# Autodesk Inventor assembly: 100-CHASSIS-ASM-01
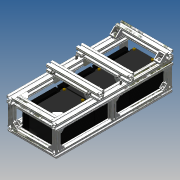
[picture p0: Inventor's stored thumbnail of the model, 180x180]
Saved by Autodesk Inventor 2018.2 (Build 222227000, 227)
## iProperties
Manager: feesmrt
Company: FRANC0R
Created: 2017-12-16
Part Number: 100-CHASSIS-ASM-01
Material: Generisch
Document SubType Name: Assembly
Designer: feesmrt
Project: Rescue Robot
Cost Center: -
Description: Chassis ASM
Engineer: feesmrt
Authority: feesmrt
Stock Number: 100-CHASSIS-ASM-01
Author: feesmrt
Title: Chassis ASM
Subject: Rescue Robot
Revision Number: 1
## Documents named in this file (3)
- D:\Programmierung\FRANC0R\CAD\02-Rocker-Bogie-Robot\100-CHASSIS\100-CHASSIS-ASM-01.iam
- D:\Programmierung\FRANC0R\CAD\02-Rocker-Bogie-Robot\100-CHASSIS\10-FRAME\100-10-FRAME-CHASSIS-ASM-01.iam
- D:\Programmierung\FRANC0R\CAD\02-Rocker-Bogie-Robot\800-ELECTRONICS\800-BATTERY-PACK.iam
## Components (2 placed, 2 different names)
1. 100-10-FRAME-CHASSIS-ASM-01:1 [sub-assembly] — Passend:1, Passend:2, Fluchtend:1
2. 800-BATTERY-PACK:1 [sub-assembly] — Passend:1, Passend:2, Fluchtend:1
## Relationships (3: Mate 2, Flush 1)
- Passend:1 [Mate] (7.5 mm): 100-10-FRAME-CHASSIS-ASM-01:1 ↔ 800-BATTERY-PACK:1
- Passend:2 [Mate]: 100-10-FRAME-CHASSIS-ASM-01:1 ↔ 800-BATTERY-PACK:1
- Fluchtend:1 [Flush]: 100-10-FRAME-CHASSIS-ASM-01:1 ↔ 800-BATTERY-PACK:1
